# Autodesk Inventor assembly: Toughbox long hex
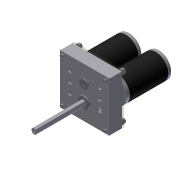
[picture p0: Inventor's stored thumbnail of the model, 180x180]
Saved by Autodesk Inventor 2011 (Build 150239000, 239)
## iProperties
Created: 2012-06-01
Part Number: Toughbox long hex
Document SubType Name: Assembly
Designer: Nemo
Mass: 3405.59 g
Surface Area: 2143.55 cm^2
Volume: 1055.37 cm^3
Density: 3.22692 g/cm^3
Author: Nemo
## Documents named in this file (15)
- H:\Nemo\Documents\Robotics\COTS Parts\Gearboxes\Toughbox Long Hex Output Shaft.iam
- H:\Nemo\Documents\Robotics\COTS Parts\Gearboxes\Housings\Toughbox Motor Plate.ipt
- H:\Nemo\Documents\Robotics\COTS Parts\Gearboxes\Bearings\Bearing FR6zz.ipt
- H:\Nemo\Documents\Robotics\COTS Parts\Gearboxes\Shafts\Toughbox Long Hex Output Shaft.ipt
- H:\Nemo\Documents\Robotics\COTS Parts\Gearboxes\Shafts\Toughbox Small Hex Shaft.ipt
- H:\Nemo\Documents\Robotics\COTS Parts\Gearboxes\Gears\Gear 20dp 375hex 50T.ipt
- H:\Nemo\Documents\Robotics\COTS Parts\Gearboxes\Gears\Gear 20dp 375hex 14T.ipt
- H:\Nemo\Documents\Robotics\COTS Parts\Gearboxes\Housings\Toughbox Enclosure.ipt
- H:\Nemo\Documents\Robotics\COTS Parts\Gearboxes\Housings\Toughbox Shaft Plate.ipt
- H:\Nemo\Documents\Robotics\COTS Parts\Gearboxes\Bearings\Bearing FR8zz-hex.ipt
- H:\Nemo\Documents\Robotics\COTS Parts\Gearboxes\Gears\Gear 20dp 500hex 50T.ipt
- H:\Nemo\Documents\Robotics\COTS Parts\Motors\CIM Motor 14T.iam
- H:\Nemo\Documents\Robotics\COTS Parts\Fasteners\10-32 SHCS x750.ipt
- H:\Nemo\Documents\Robotics\COTS Parts\Fasteners\10-32 SHCS x1750.ipt
- H:\Nemo\Documents\Robotics\COTS Parts\Fasteners\14-20 locknut.ipt
## Components (26 placed, 14 different names)
1. Toughbox Motor Plate:1 — Insert:1, Insert:2, Mate:5, Flush:1, Flush:2, Mate:6, Mate:7, Mate:11, Insert:7, Insert:8, Mate:12, Insert:9, Insert:10, Insert:11, Insert:12, Insert:17, Insert:18, Insert:19, Insert:20
2. Bearing FR6zz:1 — Insert:1, Insert:3
3. Bearing FR6zz:2 — Insert:2, Insert:4, Mate:2
4. Toughbox Long Hex Output Shaft:1 — Insert:3, Angle:3
5. Toughbox Cluster Shaft 375hex:1 — Insert:4, Mate:1, Angle:1, Mate:3, Angle:2
6. Gear 20dp 375hex 50T:1 — Mate:1, Angle:1, Mate:2, Mate:4
7. Gear 14T 20dp 375hex:1 — Mate:3, Angle:2, Mate:4
8. Toughbox Enclosure:1 — Mate:5, Flush:1, Flush:2, Mate:10
9. Toughbox Shaft Plate:1 — Insert:5, Insert:6, Mate:6, Mate:7, Mate:8, Mate:9, Mate:10, Insert:21, Insert:22, Insert:23, Insert:24
10. Bearing FR8zz-hex:1 — Insert:5
11. Bearing FR6zz:3 — Insert:6
12. Gear 50T 20dp 500hex:1 — Mate:8, Mate:9, Angle:3
13. CIM Motor 14T:1 [sub-assembly] — Insert:8, Mate:12
14. CIM Motor 14T:2 [sub-assembly] — Mate:11, Insert:7
15. 10-32 SHCS x750:1 — Insert:9
16. 10-32 SHCS x750:2 — Insert:10
17. 10-32 SHCS x750:3 — Insert:11
18. 10-32 SHCS x750:4 — Insert:12
19. 14-20 locknut:1 — Insert:19
20. 14-20 locknut:2 — Insert:17
21. 14-20 locknut:3 — Insert:20
22. 14-20 locknut:4 — Insert:18
23. 10-32 SHCS x1750:1 — Insert:24
24. 10-32 SHCS x1750:2 — Insert:23
25. 10-32 SHCS x1750:3 — Insert:22
26. 10-32 SHCS x1750:4 — Insert:21
## Relationships (37: Insert 20, Mate 12, Angle 3, Flush 2)
- Insert:1: Toughbox Motor Plate:1 ↔ Bearing FR6zz:1
- Insert:2: Toughbox Motor Plate:1 ↔ Bearing FR6zz:2
- Insert:3: Bearing FR6zz:1 ↔ Toughbox Long Hex Output Shaft:1
- Insert:4: Bearing FR6zz:2 ↔ Toughbox Cluster Shaft 375hex:1
- Mate:1: Toughbox Cluster Shaft 375hex:1 ↔ Gear 20dp 375hex 50T:1
- Angle:1 (0 deg): Toughbox Cluster Shaft 375hex:1 ↔ Gear 20dp 375hex 50T:1
- Mate:2: Bearing FR6zz:2 ↔ Gear 20dp 375hex 50T:1
- Mate:3: Toughbox Cluster Shaft 375hex:1 ↔ Gear 14T 20dp 375hex:1
- Angle:2 (0 deg): Toughbox Cluster Shaft 375hex:1 ↔ Gear 14T 20dp 375hex:1
- Mate:4: Gear 20dp 375hex 50T:1 ↔ Gear 14T 20dp 375hex:1
- Mate:5: Toughbox Motor Plate:1 ↔ Toughbox Enclosure:1
- Flush:1: Toughbox Motor Plate:1 ↔ Toughbox Enclosure:1
- Flush:2: Toughbox Motor Plate:1 ↔ Toughbox Enclosure:1
- Insert:5: Toughbox Shaft Plate:1 ↔ Bearing FR8zz-hex:1
- Insert:6: Toughbox Shaft Plate:1 ↔ Bearing FR6zz:3
- Mate:6: Toughbox Motor Plate:1 ↔ Toughbox Shaft Plate:1
- Mate:7: Toughbox Motor Plate:1 ↔ Toughbox Shaft Plate:1
- Mate:8: Toughbox Shaft Plate:1 ↔ Gear 50T 20dp 500hex:1
- Mate:9 (1.524 mm): Toughbox Shaft Plate:1 ↔ Gear 50T 20dp 500hex:1
- Angle:3 (0 deg): Toughbox Long Hex Output Shaft:1 ↔ Gear 50T 20dp 500hex:1
- Mate:10: Toughbox Enclosure:1 ↔ Toughbox Shaft Plate:1
- Mate:11: Toughbox Motor Plate:1 ↔ CIM Motor 14T:2
- Insert:7: Toughbox Motor Plate:1 ↔ CIM Motor 14T:2
- Insert:8: Toughbox Motor Plate:1 ↔ CIM Motor 14T:1
- Mate:12: Toughbox Motor Plate:1 ↔ CIM Motor 14T:1
- Insert:9: Toughbox Motor Plate:1 ↔ 10-32 SHCS x750:1
- Insert:10: Toughbox Motor Plate:1 ↔ 10-32 SHCS x750:2
- Insert:11: Toughbox Motor Plate:1 ↔ 10-32 SHCS x750:3
- Insert:12: Toughbox Motor Plate:1 ↔ 10-32 SHCS x750:4
- Insert:17: Toughbox Motor Plate:1 ↔ 14-20 locknut:2
- Insert:18: Toughbox Motor Plate:1 ↔ 14-20 locknut:4
- Insert:19: Toughbox Motor Plate:1 ↔ 14-20 locknut:1
- Insert:20: Toughbox Motor Plate:1 ↔ 14-20 locknut:3
- Insert:21: Toughbox Shaft Plate:1 ↔ 10-32 SHCS x1750:4
- Insert:22: Toughbox Shaft Plate:1 ↔ 10-32 SHCS x1750:3
- Insert:23: Toughbox Shaft Plate:1 ↔ 10-32 SHCS x1750:2
- Insert:24: Toughbox Shaft Plate:1 ↔ 10-32 SHCS x1750:1
